# Autodesk Inventor assembly: Assembly1
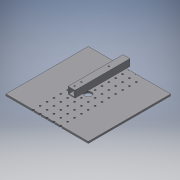
[picture p0: Inventor's stored thumbnail of the model, 180x180]
Saved by Autodesk Inventor 2018 (Build 220112000, 112)
## iProperties
Created: 2018-12-05
Part Number: Assembly1
Document SubType Name: Assembly
Designer: gbgic
Author: gbgic
## Documents named in this file (3)
- C:\Users\gbgic\Documents\Assembly1.iam
- C:\Users\gbgic\Documents\Drill Jig Base.ipt
- C:\Users\gbgic\Documents\Tube Beam.ipt
## Components (2 placed, 2 different names)
1. Drill Jig Base:1 — Mate:1, Mate:2, Mate:3
2. Tube Beam:1 — Mate:1, Mate:2, Mate:3
## Relationships (3: Mate 3)
- Mate:1: Drill Jig Base:1 ↔ Tube Beam:1
- Mate:2: Drill Jig Base:1 ↔ Tube Beam:1
- Mate:3: Drill Jig Base:1 ↔ Tube Beam:1
